# Autodesk Inventor assembly: Assembly
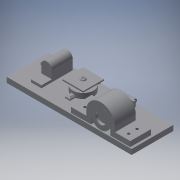
[picture p0: Inventor's stored thumbnail of the model, 180x180]
Saved by Autodesk Inventor 2016 (Build 200138000, 138)
## iProperties
Created: 2016-01-27
Part Number: Assembly
Document SubType Name: Assembly
Designer: seve
Author: seve
## Documents named in this file (8)
- C:\Users\seve\ccup\CAD\oscillator\Assembly.iam
- C:\Users\seve\ccup\CAD\dual-servo\base.ipt
- C:\Users\seve\ccup\CAD\dual-servo\solenoid.ipt
- C:\Users\seve\ccup\CAD\dual-servo\solenoid_mount.ipt
- C:\Users\seve\ccup\CAD\dual-servo\Part41.ipt
- C:\Users\seve\ccup\CAD\dual-servo\Part42.ipt
- C:\Users\seve\ccup\CAD\dual-servo\Part43.ipt
- C:\Users\seve\ccup\CAD\dual-servo\Part44.ipt
## Components (8 placed, 7 different names)
1. base:1 — Mate:1, Mate:2, Angle:1, Flush:4, Flush:5, Flush:6
2. solenoid:1 — Flush:1, Tangent:1, Tangent:2, Flush:2, Flush:3
3. solenoid_mount:1 — Flush:1, Tangent:1, Mate:2
4. solenoid_mount:2 — Tangent:2, Flush:2, Mate:1, Angle:1
5. Part41:1 — Flush:3
6. Part42:1 — Flush:4, Flush:5
7. Part43:1 — Flush:6, Flush:7
8. Part44:1 — Flush:7
## Relationships (12: Flush 7, Tangent 2, Mate 2, Angle 1)
- Flush:1: solenoid:1 ↔ solenoid_mount:1
- Tangent:1: solenoid:1 ↔ solenoid_mount:1
- Tangent:2: solenoid:1 ↔ solenoid_mount:2
- Flush:2: solenoid:1 ↔ solenoid_mount:2
- Mate:1: base:1 ↔ solenoid_mount:2
- Mate:2: base:1 ↔ solenoid_mount:1
- Angle:1 (90 deg): base:1 ↔ solenoid_mount:2
- Flush:3: solenoid:1 ↔ Part41:1
- Flush:4: base:1 ↔ Part42:1
- Flush:5: base:1 ↔ Part42:1
- Flush:6: base:1 ↔ Part43:1
- Flush:7: Part43:1 ↔ Part44:1
